# Autodesk Inventor assembly: EFOI-10
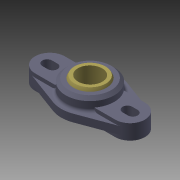
[picture p0: Inventor's stored thumbnail of the model, 180x180]
Saved by Autodesk Inventor 2014 (Build 180170000, 170)
## iProperties
Category: Plastic Bearings
Company: Autodesk, Inc.
Created: 2013-12-20
Part Number: EFOI-10
Document SubType Name: Assembly
Project: FIRST
Catalog Web Link: http://www.igus.com/wpck/5378/igubal_Flanschlager_EFOI?CL=US-en
Description: Flanged spherical bearing
Vendor: igus
Title: Flanged Spherical Bearing
Author: Autodesk, Inc.
## Documents named in this file (3)
- D:\Data Folder\FIRST 2014\KOP Parts\Plastic Bearings\PB_Bearing_EFOI-10.iam
- D:\Data Folder\FIRST 2014\KOP Parts\Plastic Bearings\Parts\EFOI-10_Housing.ipt
- D:\Data Folder\FIRST 2014\KOP Parts\Plastic Bearings\Parts\EFOI-10_Spherical Bearing.ipt
## Components (2 placed, 2 different names)
1. EFOI-10_Housing:1 — Mate:1
2. EFOI-10_Spherical Bearing:1 — Mate:1
## Relationships (1: Mate 1)
- Mate:1: EFOI-10_Housing:1 ↔ EFOI-10_Spherical Bearing:1
